# Autodesk Inventor assembly: Servo Motor
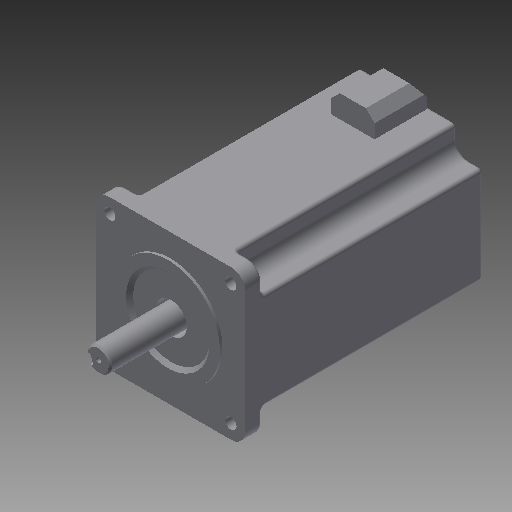
[picture p0: Inventor's stored thumbnail of the model, 512x512]
Saved by Autodesk Inventor 2018 (Build 220112000, 112)
## iProperties
Created: 2017-05-16
Part Number: Servo Motor
Document SubType Name: Assembly
Designer: M220404
Author: M220404
## Documents named in this file (3)
- C:\Users\P301319\Desktop\pack and go\Project Files\Servo Motor\Servo Motor.iam
- C:\Users\P301319\Desktop\pack and go\Project Files\Servo Motor\Body.ipt
- C:\Users\P301319\Desktop\pack and go\Project Files\Servo Motor\Shaft.ipt
## Components (2 placed, 2 different names)
1. Body:1 — Mate:1, Mate:2
2. Shaft:1 — Mate:1, Mate:2
## Relationships (2: Mate 2)
- Mate:1: Body:1 ↔ Shaft:1
- Mate:2: Body:1 ↔ Shaft:1
